# Autodesk Inventor assembly: TheClaw
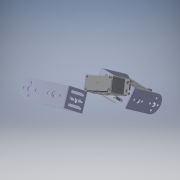
[picture p0: Inventor's stored thumbnail of the model, 180x180]
Saved by Autodesk Inventor 2017 (Build 210142000, 142)
## iProperties
Created: 2017-09-30
Part Number: TheClaw
Document SubType Name: Assembly
Designer: User
Author: User
## Documents named in this file (5)
- C:\Robotics\CAD\2017-18_CAD\TheClaw.iam
- C:\Robotics\CAD\COTSParts\Tetrix\39593_txm-standard-scale pivot armwbearing..ipt
- C:\Robotics\CAD\COTSParts\Tetrix\39020_txm-servo mount horn.ipt
- C:\Robotics\CAD\COTSParts\Tetrix\Tetrix bracket - single servo.ipt
- C:\Robotics\CAD\COTSParts\Vex\REV-41-1097.ipt
## Components (7 placed, 4 different names)
1. 39593_txm-standard-scale pivot armwbearing.:1 — Mate:16, Mate:17, Mate:18, Mate:19, Mate:20
2. 39020_txm-servo mount horn:1 — Mate:11, Mate:15, Mate:16, Mate:17, Mate:18
3. 39020_txm-servo mount horn:2 — Mate:10, Mate:19, Mate:20, Mate:21, Mate:22
4. Tetrix bracket - single servo:2 — Mate:1, Mate:2, Mate:6, Mate:14
5. REV-41-1097:2 — Mate:1, Mate:2, Mate:6, Mate:11, Mate:14, Mate:15
6. REV-41-1097:3 — Mate:10, Mate:21, Mate:22
7. 39593_txm-standard-scale pivot armwbearing.:2
## Relationships (14: Mate 14)
- Mate:1 (0.5969 mm): Tetrix bracket - single servo:2 ↔ REV-41-1097:2
- Mate:2: Tetrix bracket - single servo:2 ↔ REV-41-1097:2
- Mate:6 (4.9276 mm): Tetrix bracket - single servo:2 ↔ REV-41-1097:2
- Mate:10: 39020_txm-servo mount horn:2 ↔ REV-41-1097:3
- Mate:11: 39020_txm-servo mount horn:1 ↔ REV-41-1097:2
- Mate:14: Tetrix bracket - single servo:2 ↔ REV-41-1097:2
- Mate:15: 39020_txm-servo mount horn:1 ↔ REV-41-1097:2
- Mate:16 (3.6322 mm): 39593_txm-standard-scale pivot armwbearing.:1 ↔ 39020_txm-servo mount horn:1
- Mate:17 (3.6322 mm): 39593_txm-standard-scale pivot armwbearing.:1 ↔ 39020_txm-servo mount horn:1
- Mate:18 (3.6322 mm): 39593_txm-standard-scale pivot armwbearing.:1 ↔ 39020_txm-servo mount horn:1
- Mate:19: 39593_txm-standard-scale pivot armwbearing.:1 ↔ 39020_txm-servo mount horn:2
- Mate:20: 39593_txm-standard-scale pivot armwbearing.:1 ↔ 39020_txm-servo mount horn:2
- Mate:21: 39020_txm-servo mount horn:2 ↔ REV-41-1097:3
- Mate:22: 39020_txm-servo mount horn:2 ↔ REV-41-1097:3
